# Autodesk Inventor assembly: Assembled box
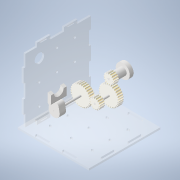
[picture p0: Inventor's stored thumbnail of the model, 180x180]
Saved by Autodesk Inventor 2021 (Build 250183000, 183)
## iProperties
Created: 2020-02-27
Part Number: Assembled box
Document SubType Name: Assembly
Designer: jstr255
Author: jstr255
## Documents named in this file (17)
- C:\Uni\Sem1\334\Project A\Final Files\Box Files\Assembled box.iam
- C:\Uni\Sem1\334\Project A\Final Files\Box Files\Box base.ipt
- C:\Uni\Sem1\334\Project A\Final Files\Box Files\Box side 1.ipt
- C:\Uni\Sem1\334\Project A\Final Files\Box Files\Box side 2.ipt
- C:\Uni\Sem1\334\Project A\Final Files\Box Files\Box side 3.ipt
- C:\Uni\Sem1\334\Project A\Final Files\Box Files\Box side 4.ipt
- C:\Uni\Sem1\334\Project A\Final Files\Box Files\Box top.ipt
- C:\Uni\Sem1\334\Project A\Final Files\ramp(2).ipt
- C:\Uni\Sem1\334\Project A\Final Files\Driveshaft coupling end.ipt
- C:\Uni\Sem1\334\Project A\Final Files\Input Connection.ipt
- C:\Uni\Sem1\334\Project A\Final Files\Final Gear Set\Design Accelerator\Final Spur Gear Large.ipt
- C:\Uni\Sem1\334\Project A\Final Files\Final Gear Set\Design Accelerator\Spur Gear12.ipt
- C:\Uni\Sem1\334\Project A\Final Files\Extra Shaft.ipt
- C:\Uni\Sem1\334\Project A\Final Files\Pear Cam.ipt
- C:\Uni\Sem1\334\Project A\Final Files\top_part.ipt
- C:\Uni\Sem1\334\Project A\Final Files\Shaft 2.ipt
- C:\Uni\Sem1\334\Project A\Final Files\Follower Ramp 2.ipt
## Components (19 placed, 16 different names)
1. Box base:1 — Mate:1, Mate:2, Mate:3, Mate:4, Mate:5, Mate:6, Mate:7, Mate:8, Mate:9, Mate:10, Flush:4, Mate:29, Mate:30
2. Box side 1:1 — Mate:1, Mate:2, Mate:3, Flush:1, Mate:14, Rotational:1
3. Box side 2:1 — Mate:4, Mate:5, Mate:6, Mate:13
4. Box side 3:1 — Mate:7, Mate:8, Mate:9, Mate:11
5. Box side 4:1 — Mate:10, Mate:11, Flush:1, Mate:12, Rigid:1, Flush:2, Mate:26, Flush:14, Flush:15, Rigid:8, Rigid:9, Flush:18
6. Box top:1 — Mate:12, Mate:13, Mate:14
7. ramp(2):1 — Rigid:1
8. Driveshaft coupling end:2 — Rotational:1, Mate:15, Mate:16, Mate:17, Angle:1
9. Input Connection:1 — Mate:15, Mate:16, Mate:17, Rigid:3
10. Spur Gear2:1 — Mate:24, Flush:11, Rotation:2, Mate:26, Rigid:5, Mate:30
11. Spur Gear1:1 — Rigid:3, Mate:24, Flush:11, Rotation:2
12. Spur Gear1:2 — Rigid:4, Flush:12, Mate:27, Rotation:3
13. Extra Shaft:1 — Rigid:4, Rigid:5
14. Spur Gear2:3 — Flush:12, Mate:27, Mate:28, Mate:29, Rotation:3, Rigid:10
15. Pear Cam:2 — Rigid:11, Flush:19, Transitional:2
16. ramp(2):2 — Rigid:8
17. top_part:1 — Rigid:9
18. Shaft 2:1 — Rigid:10, Rigid:11
19. Follower Ramp 2:1 — Flush:19, Flush:20, Transitional:2
## Relationships (46: Mate 23, Flush 10, WeldJoint 8, RelateRotation 2, RevoluteJoint 1, Angle 1, Transitional 1)
- Mate:1: Box base:1 ↔ Box side 1:1
- Mate:2: Box base:1 ↔ Box side 1:1
- Mate:3: Box base:1 ↔ Box side 1:1
- Mate:4: Box base:1 ↔ Box side 2:1
- Mate:5: Box base:1 ↔ Box side 2:1
- Mate:6: Box base:1 ↔ Box side 2:1
- Mate:7: Box base:1 ↔ Box side 3:1
- Mate:8: Box base:1 ↔ Box side 3:1
- Mate:9: Box base:1 ↔ Box side 3:1
- Mate:10: Box base:1 ↔ Box side 4:1
- Mate:11: Box side 3:1 ↔ Box side 4:1
- Flush:1: Box side 1:1 ↔ Box side 4:1
- Mate:12: Box side 4:1 ↔ Box top:1
- Mate:13: Box side 2:1 ↔ Box top:1
- Mate:14: Box side 1:1 ↔ Box top:1
- Rigid:1 [WeldJoint]: Box side 4:1 ↔ ramp(2):1
- Rotational:1 [RevoluteJoint]: Box side 1:1 ↔ Driveshaft coupling end:2
- Mate:15: Driveshaft coupling end:2 ↔ Input Connection:1
- Mate:16: Driveshaft coupling end:2 ↔ Input Connection:1
- Mate:17: Driveshaft coupling end:2 ↔ Input Connection:1
- Flush:2 (50 mm): Box side 4:1
- Rigid:3 [WeldJoint]: Input Connection:1 ↔ Spur Gear1:1
- Flush:4 (50 mm): Box base:1
- Rigid:4 [WeldJoint]: Spur Gear1:2 ↔ Extra Shaft:1
- Mate:24 (22.5 mm): Spur Gear2:1 ↔ Spur Gear1:1
- Flush:11: Spur Gear2:1 ↔ Spur Gear1:1
- Rotation:2 [RelateRotation] (0.5 ul): Spur Gear2:1 ↔ Spur Gear1:1
- Mate:26 (50 mm): Box side 4:1 ↔ Spur Gear2:1
- Rigid:5 [WeldJoint]: Spur Gear2:1 ↔ Extra Shaft:1
- Flush:12: Spur Gear1:2 ↔ Spur Gear2:3
- Mate:27 (22.5 mm): Spur Gear1:2 ↔ Spur Gear2:3
- Mate:28 (37.14 mm): Spur Gear2:3
- Mate:29 (27.147 mm): Box base:1 ↔ Spur Gear2:3
- Mate:30 (27.5 mm): Box base:1 ↔ Spur Gear2:1
- Rotation:3 [RelateRotation] (0.5 ul): Spur Gear1:2 ↔ Spur Gear2:3
- Flush:14 (27.503 mm): Box side 4:1
- Angle:1 (0 deg): Driveshaft coupling end:2
- Flush:15 (27.503 mm): Box side 4:1
- Rigid:8 [WeldJoint]: Box side 4:1 ↔ ramp(2):2
- Rigid:9 [WeldJoint]: Box side 4:1 ↔ top_part:1
- Rigid:10 [WeldJoint]: Spur Gear2:3 ↔ Shaft 2:1
- Rigid:11 [WeldJoint]: Pear Cam:2 ↔ Shaft 2:1
- Flush:18 (27.503 mm): Box side 4:1
- Flush:19 (-7.5 mm): Pear Cam:2 ↔ Follower Ramp 2:1
- Flush:20 (-2.52 mm): Follower Ramp 2:1
- Transitional:2: Pear Cam:2 ↔ Follower Ramp 2:1
